# Autodesk Inventor assembly: largeCapAssemblyGluedV01
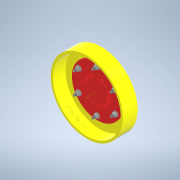
[picture p0: Inventor's stored thumbnail of the model, 180x180]
Saved by Autodesk Inventor 2021.1 (Build 251245000, 245)
## iProperties
Created: 2020-09-25
Part Number: largeCapAssemblyGluedV01
Document SubType Name: Assembly
Designer: robst
Author: robst
## Documents named in this file (7)
- C:\git\CAD-Development\robSteele\HouseProjects\Garage\CapForWater\largeCapAssemblyGluedV01.iam
- C:\git\CAD-Development\robSteele\HouseProjects\Garage\CapForWater\supportForLargeCap.ipt
- C:\git\CAD-Development\robSteele\HouseProjects\Garage\CapForWater\largeCap.ipt
- C:\Users\robst\Documents\Inventor\Content Center Files\R2021\en-US\ANSI B18.22.1\ANSI B18.22.1 - 1_4 - narrow - Type A.ipt
- C:\Users\robst\Documents\Inventor\Content Center Files\R2021\en-US\ANSI B18.21.1\ANSI B18.21.1 - 0.25.ipt
- C:\Users\robst\Documents\Inventor\Content Center Files\R2021\en-US\U UNC 2605\Unbrako - 1_4 x 1.1_4 - 20(10).ipt
- C:\Users\robst\Documents\Inventor\Content Center Files\R2021\en-US\IFI 100 107(2)\IFI 100_107 - 1_4 - 20 Metal Type.ipt
## Components (34 placed, 6 different names)
1. supportForLargeCap:1 — Flush:1, Mate:1, Mate:2, Mate:6
2. largeCap:1 — Flush:1, Mate:1, Mate:2
3. largeCap:2
4. largeCap:3 — Mate:3, Mate:4, Mate:5
5. Unbrako UNC Hex Socket Button Cap - Inch 1/4 x 1.1/4:1 — Insert:2
6. Helical Spring Lock Washers 0.25:1 — Insert:1, Insert:2
7. Plain Washer (Inch) 1/4 - narrow - Type A:1 — Mate:3, Mate:4, Insert:1
8. Plain Washer (Inch) 1/4 - narrow - Type A:2 — Mate:5, Mate:6, Insert:3
9. Prevailing Torque Type Hex Nut - Inch (IFI) 1/4 - 20 Metal Type:1 — Insert:3
10. Unbrako UNC Hex Socket Button Cap - Inch 1/4 x 1.1/4:2
11. Helical Spring Lock Washers 0.25:2
12. Plain Washer (Inch) 1/4 - narrow - Type A:3
13. Plain Washer (Inch) 1/4 - narrow - Type A:4
14. Prevailing Torque Type Hex Nut - Inch (IFI) 1/4 - 20 Metal Type:2
15. Unbrako UNC Hex Socket Button Cap - Inch 1/4 x 1.1/4:3
16. Helical Spring Lock Washers 0.25:3
17. Plain Washer (Inch) 1/4 - narrow - Type A:5
18. Plain Washer (Inch) 1/4 - narrow - Type A:6
19. Prevailing Torque Type Hex Nut - Inch (IFI) 1/4 - 20 Metal Type:3
20. Unbrako UNC Hex Socket Button Cap - Inch 1/4 x 1.1/4:4
21. Helical Spring Lock Washers 0.25:4
22. Plain Washer (Inch) 1/4 - narrow - Type A:7
23. Plain Washer (Inch) 1/4 - narrow - Type A:8
24. Prevailing Torque Type Hex Nut - Inch (IFI) 1/4 - 20 Metal Type:4
25. Unbrako UNC Hex Socket Button Cap - Inch 1/4 x 1.1/4:5
26. Helical Spring Lock Washers 0.25:5
27. Plain Washer (Inch) 1/4 - narrow - Type A:9
28. Plain Washer (Inch) 1/4 - narrow - Type A:10
29. Prevailing Torque Type Hex Nut - Inch (IFI) 1/4 - 20 Metal Type:5
30. Unbrako UNC Hex Socket Button Cap - Inch 1/4 x 1.1/4:6
31. Helical Spring Lock Washers 0.25:6
32. Plain Washer (Inch) 1/4 - narrow - Type A:11
33. Plain Washer (Inch) 1/4 - narrow - Type A:12
34. Prevailing Torque Type Hex Nut - Inch (IFI) 1/4 - 20 Metal Type:6
## Component patterns: (3 elements, first: largeCap:1), (6 elements, first: Unbrako UNC Hex Socket Button Cap - Inch 1/4 x 1.1/4:1 + Helical Spring Lock Washers 0.25:1 + Plain Washer (Inch) 1/4 - narrow - Type A:1 + Plain Washer (Inch) 1/4 - narrow - Type A:2 + Prevailing Torque Type Hex Nut - Inch (IFI) 1/4 - 20 Metal Type:1)
## Relationships (10: Mate 6, Insert 3, Flush 1)
- Flush:1: supportForLargeCap:1 ↔ largeCap:1
- Mate:1: supportForLargeCap:1 ↔ largeCap:1
- Mate:2: supportForLargeCap:1 ↔ largeCap:1
- Mate:3: largeCap:3 ↔ Plain Washer (Inch) 1/4 - narrow - Type A:1
- Mate:4: largeCap:3 ↔ Plain Washer (Inch) 1/4 - narrow - Type A:1
- Insert:1: Helical Spring Lock Washers 0.25:1 ↔ Plain Washer (Inch) 1/4 - narrow - Type A:1
- Insert:2: Unbrako UNC Hex Socket Button Cap - Inch 1/4 x 1.1/4:1 ↔ Helical Spring Lock Washers 0.25:1
- Mate:5: largeCap:3 ↔ Plain Washer (Inch) 1/4 - narrow - Type A:2
- Mate:6: supportForLargeCap:1 ↔ Plain Washer (Inch) 1/4 - narrow - Type A:2
- Insert:3: Plain Washer (Inch) 1/4 - narrow - Type A:2 ↔ Prevailing Torque Type Hex Nut - Inch (IFI) 1/4 - 20 Metal Type:1
